# Autodesk Inventor assembly: Motor Assembly
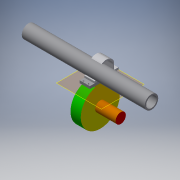
[picture p0: Inventor's stored thumbnail of the model, 180x180]
Saved by Autodesk Inventor 2016 (Build 200138000, 138)
## iProperties
Created: 2017-03-09
Part Number: Motor Assembly
Document SubType Name: Assembly
Designer: Student
Author: Student
## Documents named in this file (5)
- C:\Users\Student\Desktop\Noah Code\ROV\ROV Motor CAD Files\Motor Assembly.iam
- C:\Users\Student\Desktop\Noah Code\ROV\ROV Motor CAD Files\ROV Motor plate.ipt
- C:\Users\Student\Desktop\ROV 2-2-17\pipe clamp.ipt
- C:\Users\Student\Desktop\ROV 2-2-17\T100 rough draft.ipt
- C:\Users\Student\Desktop\Noah Code\ROV\ROV PVC Pipes\pvc pipe 1in 1ft 1.ipt
## Components (4 placed, 4 different names)
1. ROV Motor plate:1 — Rotational:1, Mate:1, Rigid:1
2. pipe clamp:1 — Rotational:1, Mate:1, Rigid:2
3. T100 rough draft:1 — Rigid:1
4. pvc pipe 1in 1ft 1:1 — Rigid:2
## Relationships (4: WeldJoint 2, RevoluteJoint 1, Mate 1)
- Rotational:1 [RevoluteJoint]: ROV Motor plate:1 ↔ pipe clamp:1
- Mate:1: ROV Motor plate:1 ↔ pipe clamp:1
- Rigid:1 [WeldJoint]: ROV Motor plate:1 ↔ T100 rough draft:1
- Rigid:2 [WeldJoint]: pipe clamp:1 ↔ pvc pipe 1in 1ft 1:1
